# Autodesk Inventor assembly: s-assy-guide_actuator
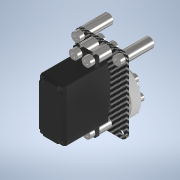
[picture p0: Inventor's stored thumbnail of the model, 180x180]
Saved by Autodesk Inventor 2022 (Build 260153000, 153)
## iProperties
Created: 2021-08-27
Part Number: s-assy-guide_actuator
Document SubType Name: Assembly
Designer: Yuta Kage
Author: Yuta Kage
## Documents named in this file (10)
- C:\Users\yuto6\Box\Public_Share\キャチロボバトルコンテスト2021\CAD\catchrobo_hardware\assy-shooter\s-assy-guide_actuator.iam
- C:\Users\yuto6\Box\Public_Share\キャチロボバトルコンテスト2021\CAD\catchrobo_hardware\assy-shooter\s_base5.ipt
- C:\Users\yuto6\Box\Public_Share\キャチロボバトルコンテスト2021\CAD\catchrobo_hardware\assy-robot\CB3-10.ipt
- C:\Users\yuto6\Box\Public_Share\キャチロボバトルコンテスト2021\CAD\catchrobo_hardware\assy-shooter\s_base6.ipt
- C:\Users\yuto6\Box\Public_Share\キャチロボバトルコンテスト2021\CAD\catchrobo_hardware\assy-shooter\SCSTR6-8.iam
- C:\Users\yuto6\Box\Public_Share\キャチロボバトルコンテスト2021\CAD\catchrobo_hardware\assy-robot\LBNR3.ipt
- C:\Users\yuto6\Box\Public_Share\キャチロボバトルコンテスト2021\CAD\catchrobo_hardware\assy-shooter\CB3-6.ipt
- C:\Users\yuto6\Box\Public_Share\キャチロボバトルコンテスト2021\CAD\catchrobo_hardware\assy-robot\ARF-420E.ipt
- C:\Users\yuto6\Box\Public_Share\キャチロボバトルコンテスト2021\CAD\catchrobo_hardware\assy-robot\CB4-6.ipt
- C:\Users\yuto6\Box\Public_Share\キャチロボバトルコンテスト2021\CAD\catchrobo_hardware\assy-shooter\s-assy-shooter_motor2.iam
## Components (34 placed, 9 different names)
1. s_base5:1 — メイト:4, メイト:5, メイト:9, メイト:13, メイト:14, メイト:15
2. s_base6:1 — メイト:6, メイト:7, メイト:9, メイト:11, メイト:12, メイト:13, メイト:16, メイト:17, メイト:39, メイト:40
3. SCSTR6-8:1 [sub-assembly] — メイト:6, メイト:7, メイト:40
4. ARF-420E:1
5. ARF-420E:2 — メイト:41, メイト:43
6. ARF-420E:3
7. CB4-6:1
8. CB4-6:2 — メイト:42
9. CB4-6:3
10. s-assy-shooter_motor2:1 [sub-assembly] — メイト:41, メイト:42, メイト:43
11. CB3-6:1 — メイト:4, メイト:5
12. CB3-10:5 — メイト:11, メイト:12
13. CB3-6:2
14. CB3-10:6
15. CB3-6:3
16. CB3-10:7
17. CB3-6:4
18. CB3-10:8
19. LBNR3:1 — メイト:14, メイト:15
20. CB3-10:9 — メイト:16, メイト:17
21. LBNR3:2
22. CB3-10:10
23. LBNR3:3
24. CB3-10:11
25. LBNR3:4
26. CB3-10:12
27. LBNR3:5
28. CB3-10:13
29. LBNR3:6
30. CB3-10:14
31. LBNR3:7
32. CB3-10:15
33. LBNR3:8
34. CB3-10:16
## Component patterns: (4 elements, first: CB3-6:1 + CB3-10:5), (8 elements, first: LBNR3:1 + CB3-10:9)
## Relationships (17: Mate 17)
- メイト:4 [Mate]: s_base5:1 ↔ CB3-6:1
- メイト:5 [Mate]: s_base5:1 ↔ CB3-6:1
- メイト:6 [Mate]: s_base6:1 ↔ SCSTR6-8:1
- メイト:7 [Mate]: s_base6:1 ↔ SCSTR6-8:1
- メイト:9 [Mate]: s_base5:1 ↔ s_base6:1
- メイト:11 [Mate]: s_base6:1 ↔ CB3-10:5
- メイト:12 [Mate]: s_base6:1 ↔ CB3-10:5
- メイト:13 [Mate]: s_base5:1 ↔ s_base6:1
- メイト:14 [Mate]: s_base5:1 ↔ LBNR3:1
- メイト:15 [Mate]: s_base5:1 ↔ LBNR3:1
- メイト:16 [Mate]: s_base6:1 ↔ CB3-10:9
- メイト:17 [Mate]: s_base6:1 ↔ CB3-10:9
- メイト:39 [Mate]: s_base6:1
- メイト:40 [Mate]: s_base6:1 ↔ SCSTR6-8:1
- メイト:41 [Mate]: ARF-420E:2 ↔ s-assy-shooter_motor2:1
- メイト:42 [Mate]: CB4-6:2 ↔ s-assy-shooter_motor2:1
- メイト:43 [Mate]: ARF-420E:2 ↔ s-assy-shooter_motor2:1
